# Autodesk Inventor assembly: Worm Gear Abstract
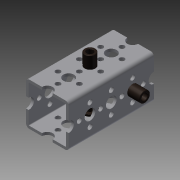
[picture p0: Inventor's stored thumbnail of the model, 180x180]
Saved by Autodesk Inventor 2015 (Build 190159000, 159)
## iProperties
Created: 2015-09-29
Part Number: Worm Gear Abstract
Document SubType Name: Assembly
Designer: Jing-Chen
Author: Jing-Chen
## Documents named in this file (3)
- C:\Users\Jing-Chen\Desktop\Bionic Hybrids 2016\Bionic-Hybrids\New Stock\Worm Gear Abstract.iam
- C:\Users\Jing-Chen\Desktop\Bionic Hybrids 2016\Bionic-Hybrids\New Stock\Worm Gear Base - 739375X108111.ipt
- C:\Users\Jing-Chen\Desktop\Bionic Hybrids 2016\Bionic-Hybrids\Stock\Bearing-Thrust - 739091.ipt
## Components (5 placed, 2 different names)
1. Worm Gear Base - 739375X108111:1 — Mate:1, Mate:2, Mate:3, Mate:4, Mate:5, Mate:6, Mate:7, Mate:8
2. Bearing-Thrust - 739091:1 — Mate:7, Mate:8
3. Bearing-Thrust - 739091:2 — Mate:2, Mate:3
4. Bearing-Thrust - 739091:3 — Mate:1, Mate:4
5. Bearing-Thrust - 739091:4 — Mate:5, Mate:6
## Relationships (8: Mate 8)
- Mate:1: Worm Gear Base - 739375X108111:1 ↔ Bearing-Thrust - 739091:3
- Mate:2: Worm Gear Base - 739375X108111:1 ↔ Bearing-Thrust - 739091:2
- Mate:3: Worm Gear Base - 739375X108111:1 ↔ Bearing-Thrust - 739091:2
- Mate:4: Worm Gear Base - 739375X108111:1 ↔ Bearing-Thrust - 739091:3
- Mate:5: Worm Gear Base - 739375X108111:1 ↔ Bearing-Thrust - 739091:4
- Mate:6: Worm Gear Base - 739375X108111:1 ↔ Bearing-Thrust - 739091:4
- Mate:7: Worm Gear Base - 739375X108111:1 ↔ Bearing-Thrust - 739091:1
- Mate:8: Worm Gear Base - 739375X108111:1 ↔ Bearing-Thrust - 739091:1
